# Autodesk Inventor assembly: Ensamblaje_eslabón
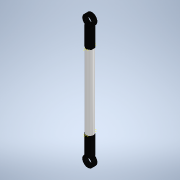
[picture p0: Inventor's stored thumbnail of the model, 180x180]
Saved by Autodesk Inventor 2020 (Build 240168000, 168)
## iProperties
Created: 2019-10-01
Part Number: Ensamblaje_eslabón
Document SubType Name: Assembly
Designer: Frederich Schnëider
Author: Frederich Schnëider
## Documents named in this file (3)
- C:\Users\Frederich Schnëider\Documents\GitHub\autobot\robot_model\Ensamblaje_eslabón.iam
- C:\Users\Frederich Schnëider\Documents\GitHub\autobot\robot_model\RCT-T003.ipt
- C:\Users\Frederich Schnëider\Documents\GitHub\autobot\robot_model\RCT-T003 (2).ipt
## Components (3 placed, 2 different names)
1. RCT-T003:1 — De rotación:1, De rotación:2
2. RCT-T003 (2):1 — De rotación:2
3. RCT-T003 (2):2 — De rotación:1
## Relationships (2: RevoluteJoint 2)
- De rotación:1 [RevoluteJoint]: RCT-T003:1 ↔ RCT-T003 (2):2
- De rotación:2 [RevoluteJoint]: RCT-T003:1 ↔ RCT-T003 (2):1
